# Autodesk Inventor assembly: assembly
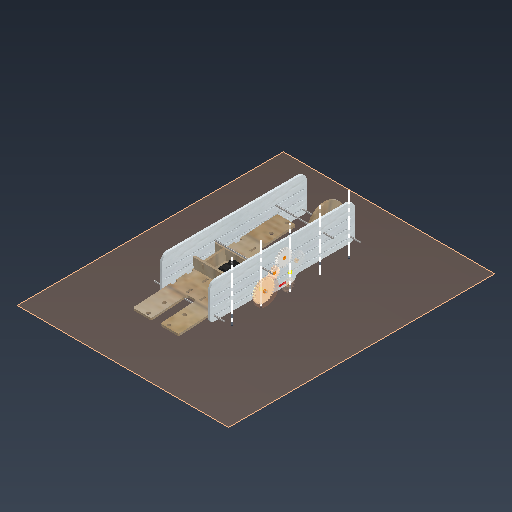
[picture p0: Inventor's stored thumbnail of the model, 512x512]
Saved by Autodesk Inventor 2025.3 (Build 293356030, 356C)
## iProperties
Created: 2025-10-01
Part Number: assembly
Document SubType Name: Assembly
Designer: 陳泓任
Author: 陳泓任
## Documents named in this file (16)
- C:\Users\Ou918\3D-model-temp\introduction to mechanical engineering(1)\version_5\assembly.iam
- C:\Users\Ou918\3D-model-temp\introduction to mechanical engineering(1)\version_5\main_frame.ipt
- C:\Users\Ou918\3D-model-temp\introduction to mechanical engineering(1)\version_5\baffle_back.ipt
- C:\Users\Ou918\3D-model-temp\introduction to mechanical engineering(1)\version_5\baffle_front.ipt
- C:\Users\Ou918\3D-model-temp\introduction to mechanical engineering(1)\version_5\support_edited.ipt
- C:\Users\Ou918\3D-model-temp\introduction to mechanical engineering(1)\version_5\bolt.ipt
- C:\Users\Ou918\3D-model-temp\introduction to mechanical engineering(1)\version_5\side_frame.ipt
- C:\Users\Ou918\3D-model-temp\introduction to mechanical engineering(1)\發條組合\發條組合.iam
- C:\Users\Ou918\3D-model-temp\introduction to mechanical engineering(1)\version_5\beam.ipt
- C:\Users\Ou918\3D-model-temp\introduction to mechanical engineering(1)\51mm wheel(with sleeve).iam
- C:\Users\Ou918\3D-model-temp\introduction to mechanical engineering(1)\100mm rod.ipt
- C:\Users\Ou918\3D-model-temp\introduction to mechanical engineering(1)\big gear(with sleeve).iam
- C:\Users\Ou918\3D-model-temp\introduction to mechanical engineering(1)\35mm wheel(with sleeve).iam
- C:\Users\Ou918\3D-model-temp\introduction to mechanical engineering(1)\sleeve.ipt
- C:\Users\Ou918\3D-model-temp\introduction to mechanical engineering(1)\small gear(with sleeve).iam
- C:\Users\Ou918\3D-model-temp\introduction to mechanical engineering(1)\middle gear.iam
## Components (22 placed, 15 different names)
1. main_frame:1 — 貼合:1, 貼合:2, 貼合:3, 貼合:4, 貼合:5, 貼合:7, 貼合:10, 貼合:11, 貼合:17, 貼合:19, 貼合:22, 貼合:24, 貼合:32, 後傾上, 前傾上, 相切:6, 相切:7, 貼合:44, 水平放置, 貼合:61, 貼合:62, 貼合:63, 貼合:64, 貼合:65, 貼合:66, 齊平:5
2. 發條組合:1 [sub-assembly] — 貼合:19, 貼合:33, 中心位置, 42mm處, 貼合:44, with gear, 貼合:47, 貼合:48, 42mm(高)
3. side_frame:1 — 齊平:1, 貼合:24, 齊平:2, 貼合:25, 齊平:3, 貼合:26, 鉛直, 側板水平, 貼合:49, 貼合:57, 貼合:58, 貼合:59, 42mm(高)
4. side_frame:2 — 齊平:1, 貼合:22, 齊平:2, 貼合:37, 貼合:39, 中心位置, 42mm處, 貼合:42, 貼合:43
5. baffle_front:1 — 貼合:4, 貼合:5, 貼合:8, 貼合:16, 貼合:32, 貼合:33
6. baffle_back:1 — 貼合:1, 貼合:2, 貼合:3
7. support_edited:1 — 貼合:7, 貼合:8, 貼合:13, 貼合:14, 貼合:16
8. support_edited:2 — 貼合:10, 貼合:11, 貼合:15, 貼合:17
9. bolt:1 — 貼合:13, 貼合:14, 貼合:15
10. beam:1 — 貼合:25, 齊平:3, 貼合:26
11. 51mm wheel(with sleeve):2 [sub-assembly] — 相切:8, 貼合:52, 貼合:66
12. 100mm rod:1 — 後傾上, 貼合:37, 貼合:52, 貼合:65
13. 100mm rod:3 — 貼合:39, 前傾上, 貼合:64
14. 100mm rod:5 — 貼合:42, 相切:6, 貼合:61, 貼合:62
15. 100mm rod:6 — 貼合:43, 相切:7, 貼合:63
16. big gear(with sleeve):1 [sub-assembly] — with gear, 貼合:46, 貼合:50
17. 35mm wheel(with sleeve):1 [sub-assembly] — 貼合:46, 貼合:47, 相切:9
18. sleeve:1 — 貼合:48, 貼合:49, 貼合:50
19. small gear(with sleeve):2 [sub-assembly] — 貼合:57, 貼合:59
20. middle gear:1 [sub-assembly] — 貼合:58
21. middle gear:2 [sub-assembly]
22. small gear(with sleeve):3 [sub-assembly]
## Relationships (59: Mate 46, Tangent 6, Flush 5, Angle 2)
- 貼合:1 [Mate]: main_frame:1 ↔ baffle_back:1
- 貼合:2 [Mate]: main_frame:1 ↔ baffle_back:1
- 貼合:3 [Mate]: main_frame:1 ↔ baffle_back:1
- 貼合:4 [Mate]: main_frame:1 ↔ baffle_front:1
- 貼合:5 [Mate]: main_frame:1 ↔ baffle_front:1
- 貼合:7 [Mate]: main_frame:1 ↔ support_edited:1
- 貼合:8 [Mate]: baffle_front:1 ↔ support_edited:1
- 貼合:10 [Mate]: main_frame:1 ↔ support_edited:2
- 貼合:11 [Mate]: main_frame:1 ↔ support_edited:2
- 貼合:13 [Mate]: support_edited:1 ↔ bolt:1
- 貼合:14 [Mate]: support_edited:1 ↔ bolt:1
- 貼合:15 [Mate]: support_edited:2 ↔ bolt:1
- 貼合:16 [Mate]: baffle_front:1 ↔ support_edited:1
- 貼合:17 [Mate]: main_frame:1 ↔ support_edited:2
- 貼合:19 [Mate]: main_frame:1 ↔ 發條組合:1
- 齊平:1 [Flush]: side_frame:1 ↔ side_frame:2
- 貼合:22 [Mate]: main_frame:1 ↔ side_frame:2
- 貼合:24 [Mate]: main_frame:1 ↔ side_frame:1
- 齊平:2 [Flush]: side_frame:1 ↔ side_frame:2
- 貼合:25 [Mate]: side_frame:1 ↔ beam:1
- 齊平:3 [Flush]: side_frame:1 ↔ beam:1
- 貼合:26 [Mate]: side_frame:1 ↔ beam:1
- 貼合:32 [Mate]: main_frame:1 ↔ baffle_front:1
- 貼合:33 [Mate]: 發條組合:1 ↔ baffle_front:1
- 後傾上 [Tangent]: main_frame:1 ↔ 100mm rod:1
- 鉛直 [Mate]: side_frame:1
- 側板水平 [Flush]: side_frame:1
- 貼合:37 [Mate]: side_frame:2 ↔ 100mm rod:1
- 貼合:39 [Mate]: side_frame:2 ↔ 100mm rod:3
- 前傾上 [Tangent]: main_frame:1 ↔ 100mm rod:3
- 中心位置 [Mate]: 發條組合:1 ↔ side_frame:2
- 42mm處 [Mate]: 發條組合:1 ↔ side_frame:2
- 貼合:42 [Mate]: side_frame:2 ↔ 100mm rod:5
- 相切:6 [Tangent]: main_frame:1 ↔ 100mm rod:5
- 貼合:43 [Mate]: side_frame:2 ↔ 100mm rod:6
- 相切:7 [Tangent]: main_frame:1 ↔ 100mm rod:6
- 貼合:44 [Mate] (-6.75 mm): main_frame:1 ↔ 發條組合:1
- with gear [Mate]: 發條組合:1 ↔ big gear(with sleeve):1
- 貼合:46 [Mate]: big gear(with sleeve):1 ↔ 35mm wheel(with sleeve):1
- 貼合:47 [Mate]: 發條組合:1 ↔ 35mm wheel(with sleeve):1
- 貼合:48 [Mate]: 發條組合:1 ↔ sleeve:1
- 貼合:49 [Mate]: side_frame:1 ↔ sleeve:1
- 貼合:50 [Mate]: big gear(with sleeve):1 ↔ sleeve:1
- 角度:1 [Angle] (0 deg)
- 相切:8 [Tangent]: 51mm wheel(with sleeve):2
- 相切:9 [Tangent]: 35mm wheel(with sleeve):1
- 水平放置 [Angle] (0 deg): main_frame:1
- 貼合:52 [Mate]: 51mm wheel(with sleeve):2 ↔ 100mm rod:1
- 貼合:57 [Mate]: side_frame:1 ↔ small gear(with sleeve):2
- 貼合:58 [Mate]: side_frame:1 ↔ middle gear:1
- 貼合:59 [Mate]: side_frame:1 ↔ small gear(with sleeve):2
- 貼合:61 [Mate]: main_frame:1 ↔ 100mm rod:5
- 貼合:62 [Mate]: main_frame:1 ↔ 100mm rod:5
- 貼合:63 [Mate]: main_frame:1 ↔ 100mm rod:6
- 貼合:64 [Mate]: main_frame:1 ↔ 100mm rod:3
- 貼合:65 [Mate]: main_frame:1 ↔ 100mm rod:1
- 貼合:66 [Mate]: main_frame:1 ↔ 51mm wheel(with sleeve):2
- 齊平:5 [Flush]: main_frame:1
- 42mm(高) [Mate]: 發條組合:1 ↔ side_frame:1
